# Autodesk Inventor assembly: Assembly6
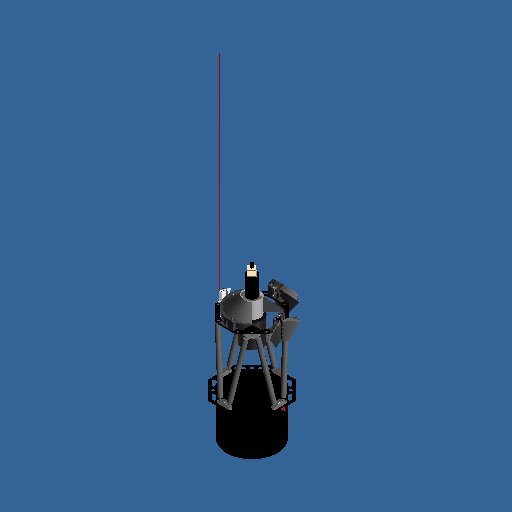
[picture p0: Inventor's stored thumbnail of the model, 512x512]
Saved by Autodesk Inventor 2026.2 (Build 302298000, 298)
## iProperties
Created: 2025-12-09
Part Number: Assembly6
Document SubType Name: Assembly
Designer: Thoma
Mass: 27295.5 g
Surface Area: 25498 cm^2
Volume: 10830.6 cm^3
Density: 2.52023 g/cm^3
Author: Thoma
## Documents named in this file (29)
- C:\Users\Thoma\OneDrive\Desktop\dir\telescope_cover\main\version_2\Main_v4.iam
- C:\Users\Thoma\OneDrive\Desktop\dir\telescope_cover\telescope\version_3\Telescope_End.ipt
- C:\Users\Thoma\OneDrive\Desktop\dir\telescope_cover\telescope\version_3\Triangle.ipt
- C:\Users\Thoma\OneDrive\Desktop\dir\telescope_cover\telescope\version_3\Triangle_Bracket_Top.ipt
- C:\Users\Thoma\OneDrive\Desktop\dir\telescope_cover\telescope\version_3\Carbon_Fibre.ipt
- C:\Users\Thoma\OneDrive\Desktop\dir\telescope_cover\telescope\version_3\5mm Screw.ipt
- C:\Users\Thoma\OneDrive\Desktop\dir\telescope_cover\telescope\version_3\35mm_bolt.ipt
- C:\Users\Thoma\OneDrive\Desktop\dir\telescope_cover\telescope\version_3\Triangle_Bracket_Bottom_MIR.ipt
- C:\Users\Thoma\OneDrive\Desktop\dir\telescope_cover\telescope\version_3\Telescope_Base.ipt
- C:\Users\Thoma\OneDrive\Desktop\dir\telescope_cover\telescope\version_3\Full_shaft_Simplify_3.ipt
- C:\Users\Thoma\OneDrive\Desktop\dir\telescope_cover\cover\Conic_Cover_Simplify_1.ipt
- C:\Users\Thoma\OneDrive\Desktop\dir\telescope_cover\telescope\version_3\30mm_bolt.ipt
- C:\Users\Thoma\OneDrive\Desktop\dir\telescope_cover\telescope\version_3\Baffle.ipt
- C:\Users\Thoma\OneDrive\Desktop\dir\telescope_cover\telescope\version_3\Bottom_End_Top.ipt
- C:\Users\Thoma\OneDrive\Desktop\dir\telescope_cover\cover\Cover_Lower_v3.ipt
- C:\Users\Thoma\OneDrive\Desktop\dir\telescope_cover\cover\Cover_Upper_v3.ipt
- C:\Users\Thoma\OneDrive\Desktop\dir\telescope_cover\telescope\version_3\4mm_0.5_Screw.ipt
- C:\Users\Thoma\OneDrive\Desktop\dir\telescope_cover\cover\Base_Plate_v2.ipt
- C:\Users\Thoma\OneDrive\Desktop\dir\telescope_cover\telescope\version_3\Laser.ipt
- C:\Users\Thoma\OneDrive\Desktop\dir\telescope_cover\cover\rod_v10.ipt
- C:\Users\Thoma\OneDrive\Desktop\dir\telescope_cover\cover\4mm_washer_1mm.ipt
- C:\Users\Thoma\OneDrive\Desktop\dir\telescope_cover\servo\DSS-M15S Servo.ipt
- C:\Users\Thoma\OneDrive\Desktop\dir\telescope_cover\cover\Base_Plate_bottom.ipt
- C:\Users\Thoma\OneDrive\Desktop\dir\telescope_cover\cover\base_plate_v5.ipt
- C:\Users\Thoma\OneDrive\Desktop\dir\telescope_cover\cover\pawn.ipt
- C:\Users\Thoma\OneDrive\Desktop\dir\telescope_cover\cover\4mm_screw.ipt
- C:\Users\Thoma\OneDrive\Desktop\dir\telescope_cover\cover\6mm_washer_1mm.ipt
- C:\Users\Thoma\OneDrive\Desktop\dir\telescope_cover\cover\casing_v3.ipt
- C:\Users\Thoma\OneDrive\Desktop\dir\telescope_cover\cover\derive_base_plate_v5.1.ipt
## Components (133 placed, 28 different names)
1. Cover_Upper_v3:1 — Tangent:38, Mate:399, Mate:400
2. Cover_Upper_v3:2 — Mate:401, Mate:402, Mate:407, Mate:408, Mate:409, Mate:410, Flush:222, Mate:418, Mate:419, Tangent:39
3. casing_v3:1 — Mate:415, Mate:416
4. rod_v10:8 — Mate:420, Mate:421, Tangent:39, Mate:422, Mate:423, Mate:428, Mate:429
5. Base_Plate_v2:1 — Mate:424, Mate:425, Mate:426, Angle:133
6. derive_base_plate_v5.1:1 — Mate:428, Mate:429, Angle:133
7. Laser:2 — Mate:214, Flush:220, Flush:221
8. Laser:1 — Mate:215, Flush:218, Flush:219
9. Baffle:1 — Mate:83
10. Carbon_Fibre:1 — Mate:7, Mate:11, Flush:1, Mate:12, Mate:13, Mate:14, Mate:15, Mate:62, Flush:2, Flush:3, Flush:4, Flush:5, Mate:83, Mate:92, Mate:93, Mate:96, Mate:97, Mate:98, Mate:99, Mate:100, Mate:123, Mate:124, Mate:125, Mate:213
11. Telescope_Base:1 — Mate:62, Angle:31, Mate:89, Mate:90, Angle:40, Mate:108, Mate:109, Angle:48, Mate:110, Mate:111, Angle:49, Mate:112, Mate:113, Angle:50, Mate:214, Mate:215, Flush:218, Flush:221
12. Telescope_End:1 — Mate:1, Mate:2, Angle:2, Mate:7, Mate:54, Mate:55, Angle:26, Angle:31, Mate:86, Mate:88, Mate:91, Angle:41, Mate:101, Angle:45, Angle:46, Mate:114, Mate:115, Angle:51, Mate:116, Mate:117, Angle:52, Mate:118, Mate:119, Angle:53, Mate:247, Mate:248, Mate:249, Mate:250, Mate:304, Mate:346, Mate:347, Mate:348, Mate:349, Mate:389, Mate:390, Mate:391, Mate:392, Mate:419, Mate:424, Mate:425, Mate:426
13. Triangle_Bracket_Top:5 — Mate:116, Mate:117, Angle:52, Mate:129, Flush:110, Angle:60
14. Triangle_Bracket_Top:4 — Mate:101, Angle:45, Angle:46, Mate:104, Mate:105, Mate:106, Flush:103, Angle:47, Angle:130
15. Triangle_Bracket_Top:3 — Mate:86, Mate:88, Mate:94, Angle:54, Angle:55, Mate:122, Flush:106, Angle:56
16. Triangle_Bracket_Top:1 — Mate:1, Mate:2, Angle:2, Mate:8, Mate:9, Angle:4, Mate:47, Angle:22, Mate:58
17. 35mm_bolt:9 — Mate:396, Mate:397, Angle:129
18. 35mm_bolt:8 — Mate:395, Mate:398, Angle:130
19. Triangle:1 — Mate:8, Mate:9, Angle:4, Mate:11, Flush:1, Angle:5, Angle:6, Mate:46, Mate:70, Mate:71
20. Triangle:5 — Mate:92, Mate:93, Mate:94, Mate:102, Mate:128, Flush:109, Angle:59, Mate:132, Flush:181, Angle:81, Flush:222
21. Triangle:6 — Mate:96, Mate:97, Mate:98, Flush:101, Angle:43, Flush:102, Angle:44, Mate:103, Mate:104, Mate:105, Mate:107
22. Triangle:7 — Mate:123, Mate:124, Mate:125, Mate:126, Flush:107, Angle:57, Mate:127, Flush:108, Angle:58, Mate:130, Mate:131
23. 35mm_bolt:6 — Mate:122, Flush:106, Angle:56
24. 35mm_bolt:7 — Mate:129, Flush:110, Angle:60
25. 35mm_bolt:4 — Mate:46, Mate:47, Angle:22
26. 35mm_bolt:5 — Mate:106, Flush:103, Angle:47
27. 5mm Screw:9 — Mate:100, Flush:102, Angle:44
28. 5mm Screw:13 — Mate:213, Flush:181, Angle:81
29. 5mm Screw:8 — Mate:99, Flush:101, Angle:43
30. 5mm Screw:10 — Mate:126, Flush:107, Angle:57
31. 5mm Screw:2 — Mate:14, Mate:15, Angle:6
32. 5mm Screw:1 — Mate:12, Mate:13, Angle:5
33. 5mm Screw:11 — Mate:127, Flush:108, Angle:58
34. 5mm Screw:12 — Mate:128, Flush:109, Angle:59
35. Full_shaft_Simplify_3:1 — Tangent:24, Tangent:25
36. Full_shaft_Simplify_3:2 — Tangent:26
37. Full_shaft_Simplify_3:3 — Tangent:27
38. Full_shaft_Simplify_3:4
39. Full_shaft_Simplify_3:5 — Tangent:29
40. Full_shaft_Simplify_3:6
41. Full_shaft_Simplify_3:7 — Tangent:32
42. Full_shaft_Simplify_3:8 — Tangent:31, Tangent:33
43. 30mm_bolt:7 — Mate:120, Flush:104, Angle:54
44. 30mm_bolt:1 — Mate:121, Flush:105, Angle:55
45. 30mm_bolt:8 — Mate:80, Flush:13, Angle:39
46. 30mm_bolt:6 — Mate:78, Flush:11, Angle:37
47. 30mm_bolt:3 — Mate:79, Flush:12, Angle:38
48. 30mm_bolt:2 — Mate:77, Flush:10, Angle:36
49. Triangle_Bracket_Bottom_MIR:4 — Mate:118, Mate:119, Angle:53, Tangent:24, Mate:395, Mate:396, Mate:397, Angle:129, Mate:398
50. Triangle_Bracket_Bottom_MIR:3 — Mate:114, Mate:115, Angle:51, Mate:120, Flush:104, Mate:121, Flush:105, Tangent:27
51. Triangle_Bracket_Bottom_MIR:2 — Mate:55, Mate:58, Angle:26, Mate:77, Flush:10, Angle:36, Mate:78, Flush:11, Angle:37, Tangent:31
52. Triangle_Bracket_Bottom_MIR:1 — Mate:54, Mate:79, Flush:12, Angle:38, Mate:80, Flush:13, Angle:39, Mate:91, Angle:41, Tangent:29, Tangent:32
53. Bottom_End_Top:4 — Mate:112, Mate:113, Angle:50, Tangent:26, Tangent:33
54. Bottom_End_Top:3 — Mate:110, Mate:111, Angle:49, Flush:219, Tangent:25
55. Bottom_End_Top:2 — Mate:108, Mate:109, Angle:48
56. Bottom_End_Top:1 — Mate:89, Mate:90, Angle:40, Flush:220
57. Conic_Cover_Simplify_1:1 — Flush:2, Mate:131, Mate:132
58. Conic_Cover_Simplify_1:2 — Flush:3, Mate:102, Mate:103, Mate:418
59. Conic_Cover_Simplify_1:3 — Flush:4, Mate:70, Mate:107
60. Conic_Cover_Simplify_1:4 — Mate:71, Flush:5, Mate:130
61. 4mm_0.5_Screw:19 — Mate:400, Mate:403, Angle:131
62. 4mm_0.5_Screw:20 — Mate:404, Mate:405
63. 4mm_0.5_Screw:21 — Mate:399, Mate:406, Angle:132
64. rod_v10:6 — Tangent:38, Mate:403, Angle:131, Mate:404, Mate:405, Mate:406, Angle:132
65. DSS-M15S Servo:3
66. Base_Plate_bottom:3 — Mate:348
67. base_plate_v5:3 — Mate:344, Mate:345, Angle:116, Mate:346, Mate:347, Mate:349
68. pawn:3
69. 6mm_washer_1mm:9
70. 6mm_washer_1mm:10
71. 6mm_washer_1mm:11
72. 6mm_washer_1mm:12
73. 4mm_screw:17
74. 4mm_screw:18
75. 4mm_screw:19
76. 4mm_screw:20
77. 4mm_screw:21
78. 4mm_screw:22
79. 4mm_screw:23
80. 4mm_screw:24 — Mate:344, Mate:345, Angle:116
81. Cover_Lower_v3:5
82. 4mm_0.5_Screw:22
83. 4mm_0.5_Screw:23
84. 4mm_0.5_Screw:24
85. rod_v10:7
86. DSS-M15S Servo:4
87. Base_Plate_bottom:4 — Mate:390
88. base_plate_v5:4 — Mate:389, Mate:391, Mate:392, Mate:393, Mate:394, Angle:128
89. pawn:4
90. 6mm_washer_1mm:13
91. 6mm_washer_1mm:14
92. 6mm_washer_1mm:15
93. 6mm_washer_1mm:16
94. 4mm_screw:25
95. 4mm_screw:26
96. 4mm_screw:27
97. 4mm_screw:28
98. 4mm_screw:29
99. 4mm_screw:30
100. 4mm_screw:31
101. 4mm_screw:32 — Mate:393, Mate:394, Angle:128
102. rod_v10:4 — Mate:216, Mate:217, Tangent:34, Mate:218, Mate:219, Mate:220, Mate:221, Mate:222, Mate:223, Mate:259, Mate:260, Angle:91
103. 4mm_washer_1mm:1 — Mate:218, Mate:219
104. 4mm_washer_1mm:2 — Mate:222, Mate:223
105. 4mm_washer_1mm:3 — Mate:220, Mate:221
106. DSS-M15S Servo:1 — Mate:228, Mate:229, Mate:230, Mate:259
107. Base_Plate_bottom:1 — Mate:250, Mate:251, Mate:252, Mate:253, Mate:254, Angle:88, Mate:255, Mate:256, Angle:89, Mate:257, Mate:258, Angle:90
108. base_plate_v5:1 — Mate:224, Mate:225, Angle:82, Mate:226, Mate:227, Angle:83, Mate:228, Mate:229, Mate:230, Mate:231, Mate:232, Mate:233, Mate:234, Mate:235, Mate:236, Mate:237, Mate:238, Mate:239, Angle:84, Mate:241, Angle:85, Mate:243, Angle:86, Angle:87, Mate:247, Mate:248, Mate:249, Mate:251, Mate:252, Angle:91
109. pawn:1 — Mate:224, Mate:225, Angle:82, Mate:260
110. 4mm_screw:1 — Mate:226, Mate:227, Angle:83
111. 6mm_washer_1mm:1 — Mate:237, Mate:238, Mate:240
112. 6mm_washer_1mm:2 — Mate:235, Mate:236, Mate:242
113. 6mm_washer_1mm:3 — Mate:233, Mate:234, Mate:245, Mate:246
114. 6mm_washer_1mm:4 — Mate:231, Mate:232, Mate:244
115. 4mm_screw:2 — Mate:239, Mate:240, Angle:84
116. 4mm_screw:3 — Mate:245, Mate:246, Angle:87
117. 4mm_screw:4 — Mate:243, Mate:244, Angle:86
118. 4mm_screw:5 — Mate:241, Mate:242, Angle:85
119. 4mm_screw:6 — Mate:255, Mate:256, Angle:89
120. 4mm_screw:7 — Mate:257, Mate:258, Angle:90
121. 4mm_screw:8 — Mate:253, Mate:254, Angle:88
122. 4mm_0.5_Screw:16 — Mate:402, Mate:407, Mate:420
123. 4mm_0.5_Screw:17 — Mate:408, Mate:409
124. 4mm_0.5_Screw:18 — Mate:401, Mate:410, Mate:421
125. DSS-M15S Servo:2 — Mate:415, Mate:416, Mate:422, Mate:423
126. Base_Plate_bottom:2 — Mate:304
127. 4mm_screw:13
128. 4mm_screw:14
129. 4mm_screw:15
130. Cover_Lower_v3:2 — Mate:207, Mate:208, Mate:209, Mate:210, Mate:211, Mate:212, Tangent:34
131. 4mm_0.5_Screw:15 — Mate:211, Mate:212, Angle:79, Mate:216
132. 4mm_0.5_Screw:14 — Mate:209, Mate:210, Angle:78, Angle:79
133. 4mm_0.5_Screw:13 — Mate:207, Mate:208, Angle:78, Mate:217
## Relationships (357: Mate 242, Angle 78, Flush 25, Tangent 12)
- Mate:1: Telescope_End:1 ↔ Triangle_Bracket_Top:1
- Mate:2: Telescope_End:1 ↔ Triangle_Bracket_Top:1
- Angle:2 (0 deg): Telescope_End:1 ↔ Triangle_Bracket_Top:1
- Mate:7: Carbon_Fibre:1 ↔ Telescope_End:1
- Mate:8: Triangle_Bracket_Top:1 ↔ Triangle:1
- Mate:9: Triangle_Bracket_Top:1 ↔ Triangle:1
- Angle:4 (0 deg): Triangle_Bracket_Top:1 ↔ Triangle:1
- Mate:11: Carbon_Fibre:1 ↔ Triangle:1
- Flush:1: Carbon_Fibre:1 ↔ Triangle:1
- Mate:12: Carbon_Fibre:1 ↔ 5mm Screw:1
- Mate:13: Carbon_Fibre:1 ↔ 5mm Screw:1
- Angle:5 (0 deg): Triangle:1 ↔ 5mm Screw:1
- Mate:14: Carbon_Fibre:1 ↔ 5mm Screw:2
- Mate:15: Carbon_Fibre:1 ↔ 5mm Screw:2
- Angle:6 (0 deg): Triangle:1 ↔ 5mm Screw:2
- Mate:46: Triangle:1 ↔ 35mm_bolt:4
- Mate:47: Triangle_Bracket_Top:1 ↔ 35mm_bolt:4
- Angle:22 (0 deg): Triangle_Bracket_Top:1 ↔ 35mm_bolt:4
- Mate:54: Telescope_End:1 ↔ Triangle_Bracket_Bottom_MIR:1
- Mate:55: Telescope_End:1 ↔ Triangle_Bracket_Bottom_MIR:2
- Mate:58: Triangle_Bracket_Top:1 ↔ Triangle_Bracket_Bottom_MIR:2
- Angle:26 (0 deg): Telescope_End:1 ↔ Triangle_Bracket_Bottom_MIR:2
- Mate:62: Carbon_Fibre:1 ↔ Telescope_Base:1
- Angle:31 (0 deg): Telescope_Base:1 ↔ Telescope_End:1
- Flush:2: Carbon_Fibre:1 ↔ Conic_Cover_Simplify_1:1
- Flush:3: Carbon_Fibre:1 ↔ Conic_Cover_Simplify_1:2
- Flush:4: Carbon_Fibre:1 ↔ Conic_Cover_Simplify_1:3
- Mate:70: Triangle:1 ↔ Conic_Cover_Simplify_1:3
- Mate:71: Triangle:1 ↔ Conic_Cover_Simplify_1:4
- Flush:5: Carbon_Fibre:1 ↔ Conic_Cover_Simplify_1:4
- Mate:77: 30mm_bolt:2 ↔ Triangle_Bracket_Bottom_MIR:2
- Flush:10: 30mm_bolt:2 ↔ Triangle_Bracket_Bottom_MIR:2
- Angle:36 (0 deg): 30mm_bolt:2 ↔ Triangle_Bracket_Bottom_MIR:2
- Mate:78: 30mm_bolt:6 ↔ Triangle_Bracket_Bottom_MIR:2
- Flush:11: 30mm_bolt:6 ↔ Triangle_Bracket_Bottom_MIR:2
- Angle:37 (0 deg): 30mm_bolt:6 ↔ Triangle_Bracket_Bottom_MIR:2
- Mate:79: 30mm_bolt:3 ↔ Triangle_Bracket_Bottom_MIR:1
- Flush:12: 30mm_bolt:3 ↔ Triangle_Bracket_Bottom_MIR:1
- Angle:38 (0 deg): 30mm_bolt:3 ↔ Triangle_Bracket_Bottom_MIR:1
- Mate:80: 30mm_bolt:8 ↔ Triangle_Bracket_Bottom_MIR:1
- Flush:13: 30mm_bolt:8 ↔ Triangle_Bracket_Bottom_MIR:1
- Angle:39 (0 deg): 30mm_bolt:8 ↔ Triangle_Bracket_Bottom_MIR:1
- Mate:83: Baffle:1 ↔ Carbon_Fibre:1
- Mate:86: Telescope_End:1 ↔ Triangle_Bracket_Top:3
- Mate:88: Telescope_End:1 ↔ Triangle_Bracket_Top:3
- Mate:89: Telescope_Base:1 ↔ Bottom_End_Top:1
- Mate:90: Telescope_Base:1 ↔ Bottom_End_Top:1
- Angle:40 (0 deg): Telescope_Base:1 ↔ Bottom_End_Top:1
- Mate:91: Telescope_End:1 ↔ Triangle_Bracket_Bottom_MIR:1
- Angle:41 (0 deg): Telescope_End:1 ↔ Triangle_Bracket_Bottom_MIR:1
- Mate:92: Carbon_Fibre:1 ↔ Triangle:5
- Mate:93: Carbon_Fibre:1 ↔ Triangle:5
- Mate:94: Triangle_Bracket_Top:3 ↔ Triangle:5
- Mate:96: Carbon_Fibre:1 ↔ Triangle:6
- Mate:97: Carbon_Fibre:1 ↔ Triangle:6
- Mate:98: Carbon_Fibre:1 ↔ Triangle:6
- Mate:99: Carbon_Fibre:1 ↔ 5mm Screw:8
- Flush:101: Triangle:6 ↔ 5mm Screw:8
- Angle:43 (0 deg): Triangle:6 ↔ 5mm Screw:8
- Mate:100: Carbon_Fibre:1 ↔ 5mm Screw:9
- Flush:102: Triangle:6 ↔ 5mm Screw:9
- Angle:44 (0 deg): Triangle:6 ↔ 5mm Screw:9
- Mate:101: Telescope_End:1 ↔ Triangle_Bracket_Top:4
- Angle:45 (0 deg): Telescope_End:1 ↔ Triangle_Bracket_Top:4
- Mate:102: Triangle:5 ↔ Conic_Cover_Simplify_1:2
- Mate:103: Triangle:6 ↔ Conic_Cover_Simplify_1:2
- Angle:46 (0 deg): Telescope_End:1 ↔ Triangle_Bracket_Top:4
- Mate:104: Triangle_Bracket_Top:4 ↔ Triangle:6
- Mate:105: Triangle_Bracket_Top:4 ↔ Triangle:6
- Mate:106: Triangle_Bracket_Top:4 ↔ 35mm_bolt:5
- Flush:103: Triangle_Bracket_Top:4 ↔ 35mm_bolt:5
- Angle:47 (0 deg): Triangle_Bracket_Top:4 ↔ 35mm_bolt:5
- Mate:107: Triangle:6 ↔ Conic_Cover_Simplify_1:3
- Mate:108: Telescope_Base:1 ↔ Bottom_End_Top:2
- Mate:109: Telescope_Base:1 ↔ Bottom_End_Top:2
- Angle:48 (0 deg): Telescope_Base:1 ↔ Bottom_End_Top:2
- Mate:110: Telescope_Base:1 ↔ Bottom_End_Top:3
- Mate:111: Telescope_Base:1 ↔ Bottom_End_Top:3
- Angle:49 (0 deg): Telescope_Base:1 ↔ Bottom_End_Top:3
- Mate:112: Telescope_Base:1 ↔ Bottom_End_Top:4
- Mate:113: Telescope_Base:1 ↔ Bottom_End_Top:4
- Angle:50 (0 deg): Telescope_Base:1 ↔ Bottom_End_Top:4
- Mate:114: Telescope_End:1 ↔ Triangle_Bracket_Bottom_MIR:3
- Mate:115: Telescope_End:1 ↔ Triangle_Bracket_Bottom_MIR:3
- Angle:51 (0 deg): Telescope_End:1 ↔ Triangle_Bracket_Bottom_MIR:3
- Mate:116: Telescope_End:1 ↔ Triangle_Bracket_Top:5
- Mate:117: Telescope_End:1 ↔ Triangle_Bracket_Top:5
- Angle:52 (0 deg): Telescope_End:1 ↔ Triangle_Bracket_Top:5
- Mate:118: Telescope_End:1 ↔ Triangle_Bracket_Bottom_MIR:4
- Mate:119: Telescope_End:1 ↔ Triangle_Bracket_Bottom_MIR:4
- Angle:53 (0 deg): Telescope_End:1 ↔ Triangle_Bracket_Bottom_MIR:4
- Mate:120: 30mm_bolt:7 ↔ Triangle_Bracket_Bottom_MIR:3
- Flush:104: 30mm_bolt:7 ↔ Triangle_Bracket_Bottom_MIR:3
- Angle:54 (0 deg): Triangle_Bracket_Top:3 ↔ 30mm_bolt:7
- Mate:121: 30mm_bolt:1 ↔ Triangle_Bracket_Bottom_MIR:3
- Flush:105: 30mm_bolt:1 ↔ Triangle_Bracket_Bottom_MIR:3
- Angle:55 (0 deg): Triangle_Bracket_Top:3 ↔ 30mm_bolt:1
- Mate:122: Triangle_Bracket_Top:3 ↔ 35mm_bolt:6
- Flush:106: Triangle_Bracket_Top:3 ↔ 35mm_bolt:6
- Angle:56 (0 deg): Triangle_Bracket_Top:3 ↔ 35mm_bolt:6
- Mate:123: Carbon_Fibre:1 ↔ Triangle:7
- Mate:124: Carbon_Fibre:1 ↔ Triangle:7
- Mate:125: Carbon_Fibre:1 ↔ Triangle:7
- Mate:126: Triangle:7 ↔ 5mm Screw:10
- Flush:107: Triangle:7 ↔ 5mm Screw:10
- Angle:57 (0 deg): Triangle:7 ↔ 5mm Screw:10
- Mate:127: Triangle:7 ↔ 5mm Screw:11
- Flush:108: Triangle:7 ↔ 5mm Screw:11
- Angle:58 (0 deg): Triangle:7 ↔ 5mm Screw:11
- Mate:128: Triangle:5 ↔ 5mm Screw:12
- Flush:109: Triangle:5 ↔ 5mm Screw:12
- Angle:59 (0 deg): Triangle:5 ↔ 5mm Screw:12
- Mate:129: Triangle_Bracket_Top:5 ↔ 35mm_bolt:7
- Flush:110: Triangle_Bracket_Top:5 ↔ 35mm_bolt:7
- Angle:60 (0 deg): Triangle_Bracket_Top:5 ↔ 35mm_bolt:7
- Mate:130: Triangle:7 ↔ Conic_Cover_Simplify_1:4
- Mate:131: Triangle:7 ↔ Conic_Cover_Simplify_1:1
- Mate:132: Triangle:5 ↔ Conic_Cover_Simplify_1:1
- Mate:207: Cover_Lower_v3:2 ↔ 4mm_0.5_Screw:13
- Mate:208: Cover_Lower_v3:2 ↔ 4mm_0.5_Screw:13
- Mate:209: Cover_Lower_v3:2 ↔ 4mm_0.5_Screw:14
- Mate:210: Cover_Lower_v3:2 ↔ 4mm_0.5_Screw:14
- Angle:78 (0 deg): 4mm_0.5_Screw:14 ↔ 4mm_0.5_Screw:13
- Mate:211: Cover_Lower_v3:2 ↔ 4mm_0.5_Screw:15
- Mate:212: Cover_Lower_v3:2 ↔ 4mm_0.5_Screw:15
- Angle:79 (0 deg): 4mm_0.5_Screw:15 ↔ 4mm_0.5_Screw:14
- Mate:213: Carbon_Fibre:1 ↔ 5mm Screw:13
- Flush:181: Triangle:5 ↔ 5mm Screw:13
- Angle:81 (0 deg): Triangle:5 ↔ 5mm Screw:13
- Mate:214: Laser:2 ↔ Telescope_Base:1
- Mate:215: Laser:1 ↔ Telescope_Base:1
- Flush:218: Laser:1 ↔ Telescope_Base:1
- Flush:219 (39.316 mm): Laser:1 ↔ Bottom_End_Top:3
- Flush:220 (39.316 mm): Laser:2 ↔ Bottom_End_Top:1
- Flush:221: Laser:2 ↔ Telescope_Base:1
- Tangent:24: Full_shaft_Simplify_3:1 ↔ Triangle_Bracket_Bottom_MIR:4
- Tangent:25: Full_shaft_Simplify_3:1 ↔ Bottom_End_Top:3
- Tangent:26: Full_shaft_Simplify_3:2 ↔ Bottom_End_Top:4
- Tangent:27: Full_shaft_Simplify_3:3 ↔ Triangle_Bracket_Bottom_MIR:3
- Tangent:29: Full_shaft_Simplify_3:5 ↔ Triangle_Bracket_Bottom_MIR:1
- Tangent:31: Full_shaft_Simplify_3:8 ↔ Triangle_Bracket_Bottom_MIR:2
- Tangent:32: Full_shaft_Simplify_3:7 ↔ Triangle_Bracket_Bottom_MIR:1
- Tangent:33: Full_shaft_Simplify_3:8 ↔ Bottom_End_Top:4
- Mate:216: rod_v10:4 ↔ 4mm_0.5_Screw:15
- Mate:217: rod_v10:4 ↔ 4mm_0.5_Screw:13
- Tangent:34 (-1 mm): rod_v10:4 ↔ Cover_Lower_v3:2
- Mate:218: rod_v10:4 ↔ 4mm_washer_1mm:1
- Mate:219: rod_v10:4 ↔ 4mm_washer_1mm:1
- Mate:220: rod_v10:4 ↔ 4mm_washer_1mm:3
- Mate:221: rod_v10:4 ↔ 4mm_washer_1mm:3
- Mate:222: rod_v10:4 ↔ 4mm_washer_1mm:2
- Mate:223: rod_v10:4 ↔ 4mm_washer_1mm:2
- Mate:224: base_plate_v5:1 ↔ pawn:1
- Mate:225: base_plate_v5:1 ↔ pawn:1
- Angle:82 (0 deg): base_plate_v5:1 ↔ pawn:1
- Mate:226: base_plate_v5:1 ↔ 4mm_screw:1
- Mate:227: base_plate_v5:1 ↔ 4mm_screw:1
- Angle:83 (0 deg): base_plate_v5:1 ↔ 4mm_screw:1
- Mate:228 (1.1 mm): DSS-M15S Servo:1 ↔ base_plate_v5:1
- Mate:229: DSS-M15S Servo:1 ↔ base_plate_v5:1
- Mate:230: DSS-M15S Servo:1 ↔ base_plate_v5:1
- Mate:231: base_plate_v5:1 ↔ 6mm_washer_1mm:4
- Mate:232: base_plate_v5:1 ↔ 6mm_washer_1mm:4
- Mate:233: base_plate_v5:1 ↔ 6mm_washer_1mm:3
- Mate:234: base_plate_v5:1 ↔ 6mm_washer_1mm:3
- Mate:235: base_plate_v5:1 ↔ 6mm_washer_1mm:2
- Mate:236: base_plate_v5:1 ↔ 6mm_washer_1mm:2
- Mate:237: base_plate_v5:1 ↔ 6mm_washer_1mm:1
- Mate:238: base_plate_v5:1 ↔ 6mm_washer_1mm:1
- Mate:239: base_plate_v5:1 ↔ 4mm_screw:2
- Mate:240: 6mm_washer_1mm:1 ↔ 4mm_screw:2
- Angle:84 (0 deg): base_plate_v5:1 ↔ 4mm_screw:2
- Mate:241: base_plate_v5:1 ↔ 4mm_screw:5
- Mate:242: 6mm_washer_1mm:2 ↔ 4mm_screw:5
- Angle:85 (0 deg): base_plate_v5:1 ↔ 4mm_screw:5
- Mate:243: base_plate_v5:1 ↔ 4mm_screw:4
- Mate:244: 6mm_washer_1mm:4 ↔ 4mm_screw:4
- Angle:86 (0 deg): base_plate_v5:1 ↔ 4mm_screw:4
- Mate:245: 6mm_washer_1mm:3 ↔ 4mm_screw:3
- Mate:246: 6mm_washer_1mm:3 ↔ 4mm_screw:3
- Angle:87 (0 deg): base_plate_v5:1 ↔ 4mm_screw:3
- Mate:247: Telescope_End:1 ↔ base_plate_v5:1
- Mate:248: Telescope_End:1 ↔ base_plate_v5:1
- Mate:249: Telescope_End:1 ↔ base_plate_v5:1
- Mate:250: Telescope_End:1 ↔ Base_Plate_bottom:1
- Mate:251: Base_Plate_bottom:1 ↔ base_plate_v5:1
- Mate:252: Base_Plate_bottom:1 ↔ base_plate_v5:1
- Mate:253: Base_Plate_bottom:1 ↔ 4mm_screw:8
- Mate:254: Base_Plate_bottom:1 ↔ 4mm_screw:8
- Angle:88 (0 deg): Base_Plate_bottom:1 ↔ 4mm_screw:8
- Mate:255: Base_Plate_bottom:1 ↔ 4mm_screw:6
- Mate:256: Base_Plate_bottom:1 ↔ 4mm_screw:6
- Angle:89 (0 deg): Base_Plate_bottom:1 ↔ 4mm_screw:6
- Mate:257: Base_Plate_bottom:1 ↔ 4mm_screw:7
- Mate:258: Base_Plate_bottom:1 ↔ 4mm_screw:7
- Angle:90 (0 deg): Base_Plate_bottom:1 ↔ 4mm_screw:7
- Mate:259: rod_v10:4 ↔ DSS-M15S Servo:1
- Mate:260 (0.57 mm): rod_v10:4 ↔ pawn:1
- Angle:91 (128.37 deg): rod_v10:4 ↔ base_plate_v5:1
- [Angle] (0 deg): 4mm_0.5_Screw:16 ↔ 4mm_0.5_Screw:17
- [Angle] (0 deg): 4mm_0.5_Screw:17 ↔ 4mm_0.5_Screw:18
- [Mate]: Base_Plate_bottom:2 ↔ 4mm_screw:15
- [Mate]: Base_Plate_bottom:2 ↔ 4mm_screw:15
- [Angle] (0 deg): Base_Plate_bottom:2 ↔ 4mm_screw:15
- [Mate]: Base_Plate_bottom:2 ↔ 4mm_screw:13
- [Mate]: Base_Plate_bottom:2 ↔ 4mm_screw:13
- [Angle] (0 deg): Base_Plate_bottom:2 ↔ 4mm_screw:13
- [Mate]: Base_Plate_bottom:2 ↔ 4mm_screw:14
- [Mate]: Base_Plate_bottom:2 ↔ 4mm_screw:14
- [Angle] (0 deg): Base_Plate_bottom:2 ↔ 4mm_screw:14
- Mate:304: Telescope_End:1 ↔ Base_Plate_bottom:2
- [Angle] (0 deg): 4mm_0.5_Screw:19 ↔ 4mm_0.5_Screw:20
- [Angle] (0 deg): 4mm_0.5_Screw:20 ↔ 4mm_0.5_Screw:21
- [Mate]: 4mm_0.5_Screw:21 ↔ rod_v10:6
- [Mate]: 4mm_0.5_Screw:19 ↔ rod_v10:6
- [Mate]: base_plate_v5:3 ↔ pawn:3
- [Mate]: base_plate_v5:3 ↔ pawn:3
- [Angle] (0 deg): base_plate_v5:3 ↔ pawn:3
- [Mate] (1.1 mm): DSS-M15S Servo:3 ↔ base_plate_v5:3
- [Mate]: DSS-M15S Servo:3 ↔ base_plate_v5:3
- [Mate]: DSS-M15S Servo:3 ↔ base_plate_v5:3
- [Mate]: base_plate_v5:3 ↔ 6mm_washer_1mm:12
- [Mate]: base_plate_v5:3 ↔ 6mm_washer_1mm:12
- [Mate]: base_plate_v5:3 ↔ 6mm_washer_1mm:11
- [Mate]: base_plate_v5:3 ↔ 6mm_washer_1mm:11
- [Mate]: base_plate_v5:3 ↔ 6mm_washer_1mm:10
- [Mate]: base_plate_v5:3 ↔ 6mm_washer_1mm:10
- [Mate]: base_plate_v5:3 ↔ 6mm_washer_1mm:9
- [Mate]: base_plate_v5:3 ↔ 6mm_washer_1mm:9
- [Mate]: base_plate_v5:3 ↔ 4mm_screw:17
- [Mate]: 6mm_washer_1mm:9 ↔ 4mm_screw:17
- [Angle] (0 deg): base_plate_v5:3 ↔ 4mm_screw:17
- [Mate]: base_plate_v5:3 ↔ 4mm_screw:20
- [Mate]: 6mm_washer_1mm:10 ↔ 4mm_screw:20
- [Angle] (0 deg): base_plate_v5:3 ↔ 4mm_screw:20
- [Mate]: base_plate_v5:3 ↔ 4mm_screw:19
- [Mate]: 6mm_washer_1mm:12 ↔ 4mm_screw:19
- [Angle] (0 deg): base_plate_v5:3 ↔ 4mm_screw:19
- [Mate]: 6mm_washer_1mm:11 ↔ 4mm_screw:18
- [Mate]: 6mm_washer_1mm:11 ↔ 4mm_screw:18
- [Angle] (0 deg): base_plate_v5:3 ↔ 4mm_screw:18
- [Mate]: Base_Plate_bottom:3 ↔ base_plate_v5:3
- [Mate]: Base_Plate_bottom:3 ↔ base_plate_v5:3
- [Mate]: Base_Plate_bottom:3 ↔ 4mm_screw:23
- [Mate]: Base_Plate_bottom:3 ↔ 4mm_screw:23
- [Angle] (0 deg): Base_Plate_bottom:3 ↔ 4mm_screw:23
- [Mate]: Base_Plate_bottom:3 ↔ 4mm_screw:21
- [Mate]: Base_Plate_bottom:3 ↔ 4mm_screw:21
- [Angle] (0 deg): Base_Plate_bottom:3 ↔ 4mm_screw:21
- [Mate]: Base_Plate_bottom:3 ↔ 4mm_screw:22
- [Mate]: Base_Plate_bottom:3 ↔ 4mm_screw:22
- [Angle] (0 deg): Base_Plate_bottom:3 ↔ 4mm_screw:22
- [Mate]: rod_v10:6 ↔ DSS-M15S Servo:3
- [Mate]: rod_v10:6 ↔ pawn:3
- [Angle] (0 deg): rod_v10:6 ↔ base_plate_v5:3
- Mate:344: base_plate_v5:3 ↔ 4mm_screw:24
- Mate:345: base_plate_v5:3 ↔ 4mm_screw:24
- Angle:116 (0 deg): base_plate_v5:3 ↔ 4mm_screw:24
- Mate:346: Telescope_End:1 ↔ base_plate_v5:3
- Mate:347: Telescope_End:1 ↔ base_plate_v5:3
- Mate:348: Telescope_End:1 ↔ Base_Plate_bottom:3
- Mate:349: Telescope_End:1 ↔ base_plate_v5:3
- [Mate]: Cover_Lower_v3:5 ↔ 4mm_0.5_Screw:22
- [Mate]: Cover_Lower_v3:5 ↔ 4mm_0.5_Screw:22
- [Mate]: Cover_Lower_v3:5 ↔ 4mm_0.5_Screw:23
- [Mate]: Cover_Lower_v3:5 ↔ 4mm_0.5_Screw:23
- [Angle] (0 deg): 4mm_0.5_Screw:22 ↔ 4mm_0.5_Screw:23
- [Mate]: Cover_Lower_v3:5 ↔ 4mm_0.5_Screw:24
- [Mate]: Cover_Lower_v3:5 ↔ 4mm_0.5_Screw:24
- [Angle] (0 deg): 4mm_0.5_Screw:23 ↔ 4mm_0.5_Screw:24
- [Mate]: 4mm_0.5_Screw:24 ↔ rod_v10:7
- [Mate]: 4mm_0.5_Screw:22 ↔ rod_v10:7
- [Tangent] (-1 mm): Cover_Lower_v3:5 ↔ rod_v10:7
- [Mate]: base_plate_v5:4 ↔ pawn:4
- [Mate]: base_plate_v5:4 ↔ pawn:4
- [Angle] (0 deg): base_plate_v5:4 ↔ pawn:4
- [Mate] (1.1 mm): DSS-M15S Servo:4 ↔ base_plate_v5:4
- [Mate]: DSS-M15S Servo:4 ↔ base_plate_v5:4
- [Mate]: DSS-M15S Servo:4 ↔ base_plate_v5:4
- [Mate]: base_plate_v5:4 ↔ 6mm_washer_1mm:16
- [Mate]: base_plate_v5:4 ↔ 6mm_washer_1mm:16
- [Mate]: base_plate_v5:4 ↔ 6mm_washer_1mm:15
- [Mate]: base_plate_v5:4 ↔ 6mm_washer_1mm:15
- [Mate]: base_plate_v5:4 ↔ 6mm_washer_1mm:14
- [Mate]: base_plate_v5:4 ↔ 6mm_washer_1mm:14
- [Mate]: base_plate_v5:4 ↔ 6mm_washer_1mm:13
- [Mate]: base_plate_v5:4 ↔ 6mm_washer_1mm:13
- [Mate]: base_plate_v5:4 ↔ 4mm_screw:25
- [Mate]: 6mm_washer_1mm:13 ↔ 4mm_screw:25
- [Angle] (0 deg): base_plate_v5:4 ↔ 4mm_screw:25
- [Mate]: base_plate_v5:4 ↔ 4mm_screw:28
- [Mate]: 6mm_washer_1mm:14 ↔ 4mm_screw:28
- [Angle] (0 deg): base_plate_v5:4 ↔ 4mm_screw:28
- [Mate]: base_plate_v5:4 ↔ 4mm_screw:27
- [Mate]: 6mm_washer_1mm:16 ↔ 4mm_screw:27
- [Angle] (0 deg): base_plate_v5:4 ↔ 4mm_screw:27
- [Mate]: 6mm_washer_1mm:15 ↔ 4mm_screw:26
- [Mate]: 6mm_washer_1mm:15 ↔ 4mm_screw:26
- [Angle] (0 deg): base_plate_v5:4 ↔ 4mm_screw:26
- [Mate]: Base_Plate_bottom:4 ↔ base_plate_v5:4
- [Mate]: Base_Plate_bottom:4 ↔ base_plate_v5:4
- [Mate]: Base_Plate_bottom:4 ↔ 4mm_screw:31
- [Mate]: Base_Plate_bottom:4 ↔ 4mm_screw:31
- [Angle] (0 deg): Base_Plate_bottom:4 ↔ 4mm_screw:31
- [Mate]: Base_Plate_bottom:4 ↔ 4mm_screw:29
- [Mate]: Base_Plate_bottom:4 ↔ 4mm_screw:29
- [Angle] (0 deg): Base_Plate_bottom:4 ↔ 4mm_screw:29
- [Mate]: Base_Plate_bottom:4 ↔ 4mm_screw:30
- [Mate]: Base_Plate_bottom:4 ↔ 4mm_screw:30
- [Angle] (0 deg): Base_Plate_bottom:4 ↔ 4mm_screw:30
- [Mate]: rod_v10:7 ↔ DSS-M15S Servo:4
- [Mate]: rod_v10:7 ↔ pawn:4
- [Angle] (0 deg): rod_v10:7 ↔ base_plate_v5:4
- Mate:389: Telescope_End:1 ↔ base_plate_v5:4
- Mate:390: Telescope_End:1 ↔ Base_Plate_bottom:4
- Mate:391: Telescope_End:1 ↔ base_plate_v5:4
- Mate:392: Telescope_End:1 ↔ base_plate_v5:4
- Mate:393: base_plate_v5:4 ↔ 4mm_screw:32
- Mate:394: base_plate_v5:4 ↔ 4mm_screw:32
- Angle:128 (0 deg): base_plate_v5:4 ↔ 4mm_screw:32
- Mate:395: 35mm_bolt:8 ↔ Triangle_Bracket_Bottom_MIR:4
- Mate:396: 35mm_bolt:9 ↔ Triangle_Bracket_Bottom_MIR:4
- Mate:397: 35mm_bolt:9 ↔ Triangle_Bracket_Bottom_MIR:4
- Angle:129 (0 deg): 35mm_bolt:9 ↔ Triangle_Bracket_Bottom_MIR:4
- Mate:398: 35mm_bolt:8 ↔ Triangle_Bracket_Bottom_MIR:4
- Angle:130 (0 deg): Triangle_Bracket_Top:4 ↔ 35mm_bolt:8
- Tangent:38 (-1 mm): Cover_Upper_v3:1 ↔ rod_v10:6
- Mate:399: Cover_Upper_v3:1 ↔ 4mm_0.5_Screw:21
- Mate:400: Cover_Upper_v3:1 ↔ 4mm_0.5_Screw:19
- Mate:401: Cover_Upper_v3:2 ↔ 4mm_0.5_Screw:18
- Mate:402: Cover_Upper_v3:2 ↔ 4mm_0.5_Screw:16
- Mate:403: 4mm_0.5_Screw:19 ↔ rod_v10:6
- Angle:131 (0 deg): 4mm_0.5_Screw:19 ↔ rod_v10:6
- Mate:404: 4mm_0.5_Screw:20 ↔ rod_v10:6
- Mate:405: 4mm_0.5_Screw:20 ↔ rod_v10:6
- Mate:406: 4mm_0.5_Screw:21 ↔ rod_v10:6
- Angle:132 (0 deg): 4mm_0.5_Screw:21 ↔ rod_v10:6
- Mate:407: Cover_Upper_v3:2 ↔ 4mm_0.5_Screw:16
- Mate:408: Cover_Upper_v3:2 ↔ 4mm_0.5_Screw:17
- Mate:409: Cover_Upper_v3:2 ↔ 4mm_0.5_Screw:17
- Mate:410: Cover_Upper_v3:2 ↔ 4mm_0.5_Screw:18
- Mate:415: casing_v3:1 ↔ DSS-M15S Servo:2
- Mate:416: casing_v3:1 ↔ DSS-M15S Servo:2
- Flush:222: Cover_Upper_v3:2 ↔ Triangle:5
- Mate:418: Cover_Upper_v3:2 ↔ Conic_Cover_Simplify_1:2
- Mate:419 (2 mm): Cover_Upper_v3:2 ↔ Telescope_End:1
- Mate:420: rod_v10:8 ↔ 4mm_0.5_Screw:16
- Mate:421: rod_v10:8 ↔ 4mm_0.5_Screw:18
- Tangent:39 (-1 mm): Cover_Upper_v3:2 ↔ rod_v10:8
- Mate:422: rod_v10:8 ↔ DSS-M15S Servo:2
- Mate:423: rod_v10:8 ↔ DSS-M15S Servo:2
- Mate:424: Base_Plate_v2:1 ↔ Telescope_End:1
- Mate:425: Base_Plate_v2:1 ↔ Telescope_End:1
- Mate:426: Base_Plate_v2:1 ↔ Telescope_End:1
- Mate:428: rod_v10:8 ↔ derive_base_plate_v5.1:1
- Mate:429: rod_v10:8 ↔ derive_base_plate_v5.1:1
- Angle:133 (180 deg): Base_Plate_v2:1 ↔ derive_base_plate_v5.1:1
## Named parameters: d715_d558 = 0 deg, d718_d561 = 0 deg, d740_d696 = 0 mm, d741_d697 = 0 mm, d742_d698 = 0 deg, d743_d699 = 0 mm, d744_d700 = 0 mm, d745_d701 = 0 deg, d746_d702 = 0 mm, d747_d703 = 0 mm, d748_d704 = 0 deg, d767_d652 = 0 mm, d768_d653 = 0 mm, d774_d558 = 0 deg, d777_d561 = 0 deg, d778_d661 = 0 mm, d779_d662 = 0 mm, d780_d663 = 0 deg, d781_d667 = 1.1 mm, d782_d668 = 0 mm, d783_d669 = 0 mm, d784_d670 = 0 mm, d785_d671 = 0 mm, d786_d672 = 0 mm, d787_d673 = 0 mm, d788_d674 = 0 mm, d789_d675 = 0 mm, d790_d676 = 0 mm, d791_d677 = 0 mm, d792_d678 = 0 mm, d793_d679 = 0 mm, d794_d680 = 0 deg, d795_d681 = 0 mm, d796_d682 = 0 mm, d797_d706 = 0 mm, d798_d707 = 0 deg, d799_d696 = 0 mm, d800_d697 = 0 mm, d801_d698 = 0 deg, d802_d699 = 0 mm, d803_d700 = 0 mm, d804_d701 = 0 deg, d805_d702 = 0 mm, d806_d703 = 0 mm, d807_d704 = 0 deg, d808_d705 = 0 mm, d809_d683 = 0 deg, d810_d684 = 0 mm, d811_d685 = 0 mm, d812_d686 = 0 deg, d813_d687 = 0 mm, d814_d688 = 0 mm, d815_d689 = 0 deg, d816_d694 = 0 mm, d817_d695 = 0 mm, d825_d652 = 0 mm, d826_d653 = 0 mm, d827_d654 = -1 mm, d828_d553 = 0 mm, d829_d554 = 0 mm, d830_d556 = 0 mm, d831_d557 = 0 mm, d832_d558 = 0 deg, d833_d559 = 0 mm, d834_d560 = 0 mm, d835_d561 = 0 deg, d836_d661 = 0 mm, d837_d662 = 0 mm, d838_d663 = 0 deg, d839_d667 = 1.1 mm, d840_d668 = 0 mm, d841_d669 = 0 mm, d842_d670 = 0 mm, d843_d671 = 0 mm, d844_d672 = 0 mm, d845_d673 = 0 mm, d846_d674 = 0 mm, d847_d675 = 0 mm, d848_d676 = 0 mm, d849_d677 = 0 mm, d850_d678 = 0 mm, d851_d679 = 0 mm, d852_d680 = 0 deg, d853_d681 = 0 mm, d854_d682 = 0 mm, d855_d706 = 0 mm, d856_d707 = 0 deg, d857_d696 = 0 mm, d858_d697 = 0 mm, d859_d698 = 0 deg, d860_d699 = 0 mm, d861_d700 = 0 mm, d862_d701 = 0 deg, d863_d702 = 0 mm, d864_d703 = 0 mm, d865_d704 = 0 deg, d866_d705 = 0 mm, d867_d683 = 0 deg, d868_d684 = 0 mm, d869_d685 = 0 mm, d870_d686 = 0 deg, d871_d687 = 0 mm, d872_d688 = 0 mm, d873_d689 = 0 deg, d874_d694 = 0 mm, d875_d695 = 0 mm
